# Autodesk Inventor assembly: Pick_&_Place_Nozzle_Assembly
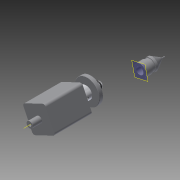
[picture p0: Inventor's stored thumbnail of the model, 180x180]
Saved by Autodesk Inventor 2015 (Build 190159000, 159)
## iProperties
Created: 2015-01-06
Part Number: Pick_&_Place_Nozzle_Assembly
Document SubType Name: Assembly
Designer: ice
Author: ice
## Documents named in this file (6)
- C:\Users\ice\Documents\GitHub\PnP-Magnetic-Tool-Tip\Inventor\Pick_&_Place_Nozzle_Assembly.iam
- C:\Users\ice\Documents\GitHub\PnP-Magnetic-Tool-Tip\Inventor\Extender.ipt
- C:\Users\ice\Documents\GitHub\PnP-Magnetic-Tool-Tip\Inventor\Nozzle#1.ipt
- C:\Users\ice\Documents\GitHub\PnP-Magnetic-Tool-Tip\Inventor\NEMA8.ipt
- C:\Users\ice\Documents\GitHub\PnP-Magnetic-Tool-Tip\Inventor\Magnet20x3x5.ipt
- C:\Users\ice\Documents\GitHub\PnP-Magnetic-Tool-Tip\Inventor\Rubber_Seal2.ipt
## Components (6 placed, 5 different names)
1. Extender:1 — Mate:4, Mate:5, Mate:10, Mate:11, Mate:12, Mate:13, Mate:14
2. Nozzle#1:1 — Mate:4
3. NEMA8:1 — Mate:5, Mate:14
4. Magnet20x3x5:1 — Mate:10, Mate:11
5. Rubber_Seal2:1 — Mate:12
6. Rubber_Seal2:2 — Mate:13
## Relationships (7: Mate 7)
- Mate:4: Extender:1 ↔ Nozzle#1:1
- Mate:5: Extender:1 ↔ NEMA8:1
- Mate:10: Extender:1 ↔ Magnet20x3x5:1
- Mate:11: Extender:1 ↔ Magnet20x3x5:1
- Mate:12: Extender:1 ↔ Rubber_Seal2:1
- Mate:13: Extender:1 ↔ Rubber_Seal2:2
- Mate:14: Extender:1 ↔ NEMA8:1
